# Autodesk Inventor assembly: Montagem traseiro
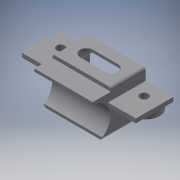
[picture p0: Inventor's stored thumbnail of the model, 180x180]
Saved by Autodesk Inventor 2019 (Build 230136000, 136)
## iProperties
Created: 2021-06-28
Part Number: Montagem traseiro
Material: Genérico
Document SubType Name: Assembly
Designer: SOU O MELHOR
Author: SOU O MELHOR
## Documents named in this file (4)
- F:\Lucas\BAJA\Inventor\Atividades\Nova fixação do acelerometro 2\Montagem traseiro.iam
- F:\Lucas\BAJA\Inventor\Atividades\Nova fixação do acelerometro 2\Caixa traseira.ipt
- F:\Lucas\BAJA\Inventor\Atividades\Nova fixação do acelerometro 2\Fixador traseiro.ipt
- C:\Users\SOU O MELHOR\Documents\Inventor\Content Center Files\R2019\pt-BR\AS 1474(1)\AS 1474 - M3(1).ipt
## Components (4 placed, 3 different names)
1. Caixa traseira:1 — Coincidência:1, Coincidência:2, Inserir:1, Inserir:2
2. Fixador traseiro:1 — Coincidência:1, Coincidência:2
3. AS 1474 - Métrica M3:1 — Inserir:1
4. AS 1474 - Métrica M3:2 — Inserir:2
## Relationships (4: Mate 2, Insert 2)
- Coincidência:1 [Mate]: Caixa traseira:1 ↔ Fixador traseiro:1
- Coincidência:2 [Mate]: Caixa traseira:1 ↔ Fixador traseiro:1
- Inserir:1: Caixa traseira:1 ↔ AS 1474 - Métrica M3:1
- Inserir:2: Caixa traseira:1 ↔ AS 1474 - Métrica M3:2
